# Autodesk Inventor assembly: Hinge
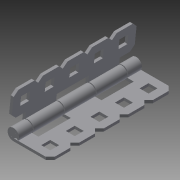
[picture p0: Inventor's stored thumbnail of the model, 180x180]
Saved by Autodesk Inventor 2015 SP1 (Build 190203100, 203)
## iProperties
Created: 2014-04-01
Part Number: Hinge
Document SubType Name: Assembly
Designer: Chris
Author: Chris
## Documents named in this file (4)
- D:\Users\Christopher\Google Drive\VEX CAD Library\Gussets\Hinge.iam
- D:\Users\Christopher\Google Drive\VEX CAD Library\Gussets\Hinge Plate 2.ipt
- D:\Users\Christopher\Google Drive\VEX CAD Library\Gussets\Hinge Pin.ipt
- D:\Users\Christopher\Google Drive\VEX CAD Library\Gussets\Hinge Plate 1.ipt
## Components (3 placed, 3 different names)
1. Hinge Plate 2:1 — Mate:2, Mate:3
2. Hinge Pin:1 — Mate:1, Mate:2, Flush:1
3. Hinge Plate 1:1 — Mate:1, Flush:1, Mate:3
## Relationships (4: Mate 3, Flush 1)
- Mate:1: Hinge Pin:1 ↔ Hinge Plate 1:1
- Mate:2: Hinge Plate 2:1 ↔ Hinge Pin:1
- Flush:1: Hinge Pin:1 ↔ Hinge Plate 1:1
- Mate:3 (0.381 mm): Hinge Plate 2:1 ↔ Hinge Plate 1:1
